# Autodesk Inventor assembly: SUBWashChamber
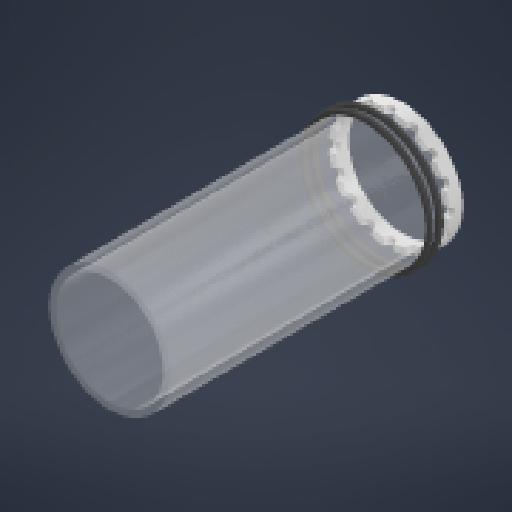
[picture p0: Inventor's stored thumbnail of the model, 512x512]
Saved by Autodesk Inventor 2024 (Build 280153000, 153)
## iProperties
Created: 2025-02-06
Part Number: SUBWashChamber
Document SubType Name: Assembly
Designer: Tommy Rohmann
Author: Tommy Rohmann
## Documents named in this file (6)
- C:\Users\Tommy Rohmann\OneDrive\Projects\Microgravity-Press-Washing-Machine\System Design and Documentation\Inventor Design Project\SUBWashChamber.iam
- C:\Users\Tommy Rohmann\OneDrive\Projects\Microgravity-Press-Washing-Machine\System Design and Documentation\Inventor Design Project\LAYOUT.ipt
- C:\Users\Tommy Rohmann\OneDrive\Projects\Microgravity-Press-Washing-Machine\System Design and Documentation\Inventor Design Project\WashChamber.ipt
- C:\Users\Tommy Rohmann\OneDrive\Projects\Microgravity-Press-Washing-Machine\System Design and Documentation\Inventor Design Project\ConduitStaticSeal.ipt
- C:\Users\Tommy Rohmann\OneDrive\Projects\Microgravity-Press-Washing-Machine\System Design and Documentation\Inventor Design Project\CastleSpacer.ipt
- C:\Users\Tommy Rohmann\OneDrive\Projects\Microgravity-Press-Washing-Machine\System Design and Documentation\Inventor Design Project\WashChamberConduit_1.ipt
## Components (6 placed, 5 different names)
1. LAYOUT:1
2. WashChamber:1 — Mate:6
3. ConduitStaticSeal:1
4. ConduitStaticSeal:2
5. CastleSpacer:1 — Mate:6
6. WashChamberConduit:1
## Relationships (4: Composite 3, Mate 1)
- [Composite]: LAYOUT:1 ↔ WashChamber:1
- [Composite]: LAYOUT:1 ↔ CastleSpacer:1
- Mate:6: WashChamber:1 ↔ CastleSpacer:1
- [Composite]: LAYOUT:1 ↔ WashChamberConduit:1
